# Autodesk Inventor assembly: SeederAssembly
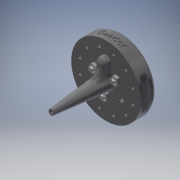
[picture p0: Inventor's stored thumbnail of the model, 180x180]
Saved by Autodesk Inventor 2017 (Build 210142000, 142)
## iProperties
Created: 2017-01-03
Part Number: SeederAssembly
Document SubType Name: Assembly
Designer: umr
Author: umr
## Documents named in this file (3)
- D:\SeniorProject\Models2\HeadTools\SeederAssembly.iam
- D:\SeniorProject\Models2\HeadTools\Seeder.ipt
- D:\SeniorProject\Models2\HeadTools\MagnetAssembly.iam
## Components (4 placed, 2 different names)
1. Seeder:1 — Mate:1, Mate:2
2. MagnetAssembly:3 [sub-assembly] — Mate:1, Mate:2
3. MagnetAssembly:4 [sub-assembly]
4. MagnetAssembly:5 [sub-assembly]
## Component patterns: (3 elements, first: MagnetAssembly:3)
## Relationships (2: Mate 2)
- Mate:1: Seeder:1 ↔ MagnetAssembly:3
- Mate:2: Seeder:1 ↔ MagnetAssembly:3
